# Autodesk Inventor assembly: silothingassem
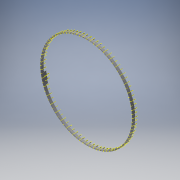
[picture p0: Inventor's stored thumbnail of the model, 180x180]
Saved by Autodesk Inventor 2019 (Build 230136000, 136)
## iProperties
Created: 2018-07-21
Part Number: silothingassem
Document SubType Name: Assembly
Designer: Kitte_X
Author: Kitte_X
## Documents named in this file (3)
- C:\Users\Kitte_X\Documents\Inventor\silothingassem.iam
- C:\Users\Kitte_X\Documents\Inventor\silothingp1.ipt
- C:\Users\Kitte_X\Documents\Inventor\silothingp2.ipt
## Components (86 placed, 2 different names)
1. silothingp1:43
2. silothingp2:43 — Mate:1, Mate:2
3. silothingp2:1 — Flush:1, Tangent:1, Flush:2
4. silothingp1:1 — Flush:1, Tangent:1, Flush:2
5. silothingp2:2 — Mate:1, Mate:2
6. silothingp1:2
7. silothingp2:3
8. silothingp1:3
9. silothingp2:4
10. silothingp1:4
11. silothingp2:5
12. silothingp1:5
13. silothingp2:6
14. silothingp1:6
15. silothingp2:7
16. silothingp1:7
17. silothingp2:8
18. silothingp1:8
19. silothingp2:9
20. silothingp1:9
21. silothingp2:10
22. silothingp1:10
23. silothingp2:11
24. silothingp1:11
25. silothingp2:12
26. silothingp1:12
27. silothingp2:13
28. silothingp1:13
29. silothingp2:14
30. silothingp1:14
31. silothingp2:15
32. silothingp1:15
33. silothingp2:16
34. silothingp1:16
35. silothingp2:17
36. silothingp1:17
37. silothingp2:18
38. silothingp1:18
39. silothingp2:19
40. silothingp1:19
41. silothingp2:20
42. silothingp1:20
43. silothingp2:21
44. silothingp1:21
45. silothingp2:22
46. silothingp1:22
47. silothingp2:23
48. silothingp1:23
49. silothingp2:24
50. silothingp1:24
51. silothingp2:25
52. silothingp1:25
53. silothingp2:26
54. silothingp1:26
55. silothingp2:27
56. silothingp1:27
57. silothingp2:28
58. silothingp1:28
59. silothingp2:29
60. silothingp1:29
61. silothingp2:30
62. silothingp1:30
63. silothingp2:31
64. silothingp1:31
65. silothingp2:32
66. silothingp1:32
67. silothingp2:33
68. silothingp1:33
69. silothingp2:34
70. silothingp1:34
71. silothingp2:35
72. silothingp1:35
73. silothingp2:36
74. silothingp1:36
75. silothingp2:37
76. silothingp1:37
77. silothingp2:38
78. silothingp1:38
79. silothingp2:39
80. silothingp1:39
81. silothingp2:40
82. silothingp1:40
83. silothingp2:41
84. silothingp1:41
85. silothingp2:42
86. silothingp1:42
## Component patterns: (42 elements, first: silothingp2:1 + silothingp1:1)
## Relationships (8: Flush 4, Tangent 2, Mate 2)
- Flush:1: silothingp2:1 ↔ silothingp1:1
- Tangent:1: silothingp2:1 ↔ silothingp1:1
- Flush:2: silothingp2:1 ↔ silothingp1:1
- [Flush]: silothingp1:43 ↔ silothingp2:43
- [Tangent]: silothingp1:43 ↔ silothingp2:43
- [Flush]: silothingp1:43 ↔ silothingp2:43
- Mate:1: silothingp2:43 ↔ silothingp2:2
- Mate:2: silothingp2:43 ↔ silothingp2:2
## Named parameters: d10_d0 = 0 mm, d11_d1 = 0 mm, d12_d2 = 0 mm
